# Autodesk Inventor assembly: JHeadmkV
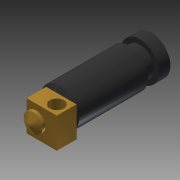
[picture p0: Inventor's stored thumbnail of the model, 180x180]
Saved by Autodesk Inventor 2015 (Build 190159000, 159)
## iProperties
Created: 2014-08-19
Part Number: JHeadmkV
Document SubType Name: Assembly
Designer: t_clevj
Author: t_clevj
## Documents named in this file (3)
- C:\Users\Jack\ownCloud\Projects\CoreXY\InventorModel\HotEnds\JHeadmkV\JHeadmkV.iam
- C:\Users\Jack\ownCloud\Projects\CoreXY\InventorModel\HotEnds\JHeadmkV\JHeadNozzle.ipt
- C:\Users\Jack\ownCloud\Projects\CoreXY\InventorModel\HotEnds\JHeadmkV\JHeadNozzleHolder.ipt
## Components (2 placed, 2 different names)
1. JHeadNozzle:1 — Mate:1, Mate:2, Mate:3, Flush:1, Mate:4
2. JHeadNozzleHolder:1 — Mate:1, Mate:2
## Relationships (5: Mate 4, Flush 1)
- Mate:1: JHeadNozzle:1 ↔ JHeadNozzleHolder:1
- Mate:2: JHeadNozzle:1 ↔ JHeadNozzleHolder:1
- Mate:3: JHeadNozzle:1
- Flush:1: JHeadNozzle:1
- Mate:4: JHeadNozzle:1
